# Autodesk Inventor assembly: laserAssemblyFull
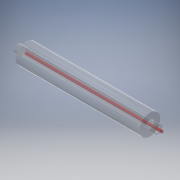
[picture p0: Inventor's stored thumbnail of the model, 180x180]
Saved by Autodesk Inventor 2017 SP1 (Build 210196100, 196)
## iProperties
Created: 2018-09-19
Part Number: laserAssemblyFull
Document SubType Name: Assembly
Designer: Sam
Author: Sam
## Documents named in this file (3)
- C:\Users\Sam\Documents\Inventor\outreach\michelson2016\inventor\laserAssemblyFull.iam
- C:\Users\Sam\Documents\Inventor\outreach\michelson2016\inventor\laserbody.ipt
- C:\Users\Sam\Documents\Inventor\outreach\michelson2016\inventor\beam small 101.ipt
## Components (2 placed, 2 different names)
1. laserbody:1 — Insert:1
2. beam small 101:1 — Insert:1
## Relationships (1: Insert 1)
- Insert:1 (-5 mm): laserbody:1 ↔ beam small 101:1
